# Autodesk Inventor assembly: КВ33.044.000
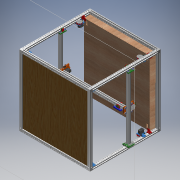
[picture p0: Inventor's stored thumbnail of the model, 180x180]
Saved by Autodesk Inventor 2019 (Build 230136000, 136)
## iProperties
Created: 2019-07-15
Part Number: КВ33.044.000
Material: Типовые
Document SubType Name: Assembly
Designer: Петров Иван
Description: Сортирующая ячейка
Author: Петров Иван
## Documents named in this file (14)
- E:\IVAN\Kvantoriada2019\optimal_gripper\hardware\КВ33.044.000 - Сортирующая ячейка.iam
- E:\IVAN\Kvantoriada2019\optimal_gripper\hardware\Стандартные изделия\Профиль станочный 30x30x740.ipt
- E:\IVAN\Kvantoriada2019\optimal_gripper\hardware\Стандартные изделия\Угол соединительный 30х30х30.ipt
- E:\IVAN\Kvantoriada2019\optimal_gripper\hardware\КВ33.044.001 - Дно.ipt
- E:\IVAN\Kvantoriada2019\optimal_gripper\hardware\КВ33.044.700 - Сборка деражтеля катка 6 мм.iam
- E:\IVAN\Kvantoriada2019\optimal_gripper\hardware\КВ33.044.400 -  Сборка сервомотора Dynamixel с крепление.iam
- E:\IVAN\Kvantoriada2019\optimal_gripper\hardware\КВ33.044.500 -  Сборка сервомотора Dynamixel с крепление обратный.iam
- E:\IVAN\Kvantoriada2019\optimal_gripper\hardware\КВ33.044.200 - Каретка оси Z.iam
- E:\IVAN\Kvantoriada2019\optimal_gripper\hardware\Стандартные изделия\Профиль станочный 30x30x717.ipt
- E:\IVAN\Kvantoriada2019\optimal_gripper\hardware\КВ33.044.300 - Каретка оси X.iam
- E:\IVAN\Kvantoriada2019\optimal_gripper\hardware\КВ33.044.003 - крепеж дна блока управления.ipt
- E:\IVAN\Kvantoriada2019\optimal_gripper\hardware\КВ33.044.100 - Блок управления.iam
- E:\IVAN\Kvantoriada2019\optimal_gripper\hardware\КВ33.044.005 - Крышка блока управления.ipt
- E:\IVAN\Kvantoriada2019\optimal_gripper\hardware\КВ33.044.600 - Каретка оси Y.iam
## Components (45 placed, 13 different names)
1. КВ33.044.001 - Дно:1 — Совмещение:65, Совмещение:66, Совмещение:67
2. Профиль станочный 30x30x740:1 — Заподлицо:9, Заподлицо:10, Совмещение:4, Заподлицо:12, Совмещение:9, Заподлицо:17
3. Профиль станочный 30x30x740:2 — Совмещение:3, Заподлицо:2, Заподлицо:3, Совмещение:66, Совмещение:67, Совмещение:105
4. Профиль станочный 30x30x740:3 — Совмещение:1, Заподлицо:1, Заподлицо:5, Заподлицо:6, Заподлицо:8, Совмещение:5, Совмещение:65, Совмещение:109
5. Профиль станочный 30x30x740:4 — Заподлицо:14, Совмещение:7, Заподлицо:16, Заподлицо:18, Заподлицо:19, Совмещение:10, Совмещение:100, Совмещение:113
6. Угол соединительный 30х30х30:1 — Совмещение:1, Совмещение:2, Совмещение:3, Заподлицо:1, Заподлицо:2, Заподлицо:3, Заподлицо:4, Заподлицо:5, Заподлицо:38
7. Угол соединительный 30х30х30:2 — Заподлицо:18, Заподлицо:19, Совмещение:10, Совмещение:11, Заподлицо:20, Заподлицо:21
8. Угол соединительный 30х30х30:3 — Заподлицо:6, Заподлицо:7, Заподлицо:8, Заподлицо:9, Заподлицо:10, Совмещение:4, Заподлицо:11, Совмещение:5, Совмещение:6
9. Угол соединительный 30х30х30:4 — Заподлицо:12, Заподлицо:13, Заподлицо:14, Заподлицо:15, Совмещение:7, Совмещение:8, Заподлицо:16, Совмещение:9, Заподлицо:17
10. Профиль станочный 30x30x740:9 — Заподлицо:7, Заподлицо:11, Совмещение:6, Совмещение:19, Заподлицо:36, Заподлицо:37, Совмещение:108, Заподлицо:46, Совмещение:139, Заподлицо:57, Совмещение:146, Совмещение:147, Совмещение:164, Совмещение:165
11. Профиль станочный 30x30x740:10 — Заподлицо:13, Заподлицо:15, Совмещение:8, Совмещение:112, Заподлицо:48, Совмещение:140, Заподлицо:58, Совмещение:148, Совмещение:149, Совмещение:173, Совмещение:175
12. Профиль станочный 30x30x740:11 — Совмещение:11, Заподлицо:20, Заподлицо:21, Совмещение:101, Заподлицо:42, Совмещение:134, Заподлицо:55, Совмещение:142, Совмещение:143, Совмещение:167, Совмещение:169
13. Профиль станочный 30x30x740:12 — Совмещение:2, Заподлицо:4, Заподлицо:38, Совмещение:104, Заподлицо:44, Совмещение:136, Заподлицо:56, Совмещение:144, Совмещение:145, Совмещение:170, Совмещение:171
14. Профиль станочный 30x30x740:15 — Совмещение:138, Совмещение:141
15. Профиль станочный 30x30x740:16 — Совмещение:135, Совмещение:137, Совмещение:177, Совмещение:179
16. Профиль станочный 30x30x740:17
17. Профиль станочный 30x30x740:18 — Совмещение:178, Совмещение:180
18. Угол соединительный 30х30х30:5
19. Угол соединительный 30х30х30:6
20. Угол соединительный 30х30х30:7 — Совмещение:19, Заподлицо:36, Заподлицо:37
21. Угол соединительный 30х30х30:8
22. КВ33.044.700 - Сборка деражтеля катка 6 мм:6 [sub-assembly] — Совмещение:100, Совмещение:101, Заподлицо:42
23. КВ33.044.700 - Сборка деражтеля катка 6 мм:7 [sub-assembly] — Совмещение:104, Заподлицо:44, Совмещение:105
24. КВ33.044.700 - Сборка деражтеля катка 6 мм:9 [sub-assembly] — Совмещение:108, Совмещение:109, Заподлицо:46
25. КВ33.044.700 - Сборка деражтеля катка 6 мм:10 [sub-assembly] — Совмещение:112, Заподлицо:48, Совмещение:113
26. КВ33.044.400 -  Сборка сервомотора Dynamixel с крепление:1 [sub-assembly] — Совмещение:134, Совмещение:135, Заподлицо:55, Совмещение:168
27. КВ33.044.500 -  Сборка сервомотора Dynamixel с крепление обратный:1 [sub-assembly] — Совмещение:136, Совмещение:137, Заподлицо:56, Совмещение:172
28. КВ33.044.400 -  Сборка сервомотора Dynamixel с крепление:2 [sub-assembly] — Совмещение:138, Совмещение:139, Заподлицо:57, Совмещение:166
29. КВ33.044.500 -  Сборка сервомотора Dynamixel с крепление обратный:2 [sub-assembly] — Совмещение:140, Заподлицо:58, Совмещение:141, Совмещение:174
30. КВ33.044.200 - Каретка оси Z:1 [sub-assembly] — Совмещение:142, Совмещение:143, Совмещение:152, Совмещение:153
31. КВ33.044.200 - Каретка оси Z:2 [sub-assembly] — Совмещение:148, Совмещение:149, Совмещение:156, Совмещение:157
32. КВ33.044.200 - Каретка оси Z:3 [sub-assembly] — Совмещение:146, Совмещение:147, Совмещение:154, Совмещение:155
33. КВ33.044.200 - Каретка оси Z:4 [sub-assembly] — Совмещение:144, Совмещение:145, Совмещение:150, Совмещение:151
34. Профиль станочный 30x30x717:1 — Совмещение:150, Совмещение:151, Совмещение:152, Совмещение:153, Совмещение:159, Заподлицо:60
35. Профиль станочный 30x30x717:2 — Совмещение:154, Совмещение:155, Совмещение:156, Совмещение:157, Совмещение:158, Заподлицо:59
36. КВ33.044.300 - Каретка оси X:1 [sub-assembly] — Совмещение:158, Заподлицо:59, Совмещение:163
37. КВ33.044.300 - Каретка оси X:2 [sub-assembly] — Совмещение:159, Заподлицо:60, Совмещение:160, Совмещение:161, Совмещение:162
38. Профиль станочный 30x30x717:3 — Совмещение:160, Совмещение:161, Совмещение:162, Совмещение:163, Совмещение:181, Совмещение:182
39. КВ33.044.003 - крепеж дна блока управления:1 — Совмещение:164, Совмещение:165, Совмещение:166
40. КВ33.044.003 - крепеж дна блока управления:2 — Совмещение:173, Совмещение:174, Совмещение:175
41. КВ33.044.003 - крепеж дна блока управления:3 — Совмещение:167, Совмещение:168, Совмещение:169
42. КВ33.044.003 - крепеж дна блока управления:4 — Совмещение:170, Совмещение:171, Совмещение:172, Совмещение:176
43. КВ33.044.100 - Блок управления:1 [sub-assembly] — Совмещение:176, Совмещение:177, Совмещение:178
44. КВ33.044.005 - Крышка блока управления:1 — Совмещение:179, Совмещение:180
45. КВ33.044.600 - Каретка оси Y:1 [sub-assembly] — Совмещение:181, Совмещение:182
## Relationships (127: Mate 79, Flush 48)
- Совмещение:1 [Mate]: Профиль станочный 30x30x740:3 ↔ Угол соединительный 30х30х30:1
- Совмещение:2 [Mate]: Угол соединительный 30х30х30:1 ↔ Профиль станочный 30x30x740:12
- Совмещение:3 [Mate]: Профиль станочный 30x30x740:2 ↔ Угол соединительный 30х30х30:1
- Заподлицо:1 [Flush]: Профиль станочный 30x30x740:3 ↔ Угол соединительный 30х30х30:1
- Заподлицо:2 [Flush]: Профиль станочный 30x30x740:2 ↔ Угол соединительный 30х30х30:1
- Заподлицо:3 [Flush]: Профиль станочный 30x30x740:2 ↔ Угол соединительный 30х30х30:1
- Заподлицо:4 [Flush]: Угол соединительный 30х30х30:1 ↔ Профиль станочный 30x30x740:12
- Заподлицо:5 [Flush]: Профиль станочный 30x30x740:3 ↔ Угол соединительный 30х30х30:1
- Заподлицо:6 [Flush]: Профиль станочный 30x30x740:3 ↔ Угол соединительный 30х30х30:3
- Заподлицо:7 [Flush]: Угол соединительный 30х30х30:3 ↔ Профиль станочный 30x30x740:9
- Заподлицо:8 [Flush]: Профиль станочный 30x30x740:3 ↔ Угол соединительный 30х30х30:3
- Заподлицо:9 [Flush]: Профиль станочный 30x30x740:1 ↔ Угол соединительный 30х30х30:3
- Заподлицо:10 [Flush]: Профиль станочный 30x30x740:1 ↔ Угол соединительный 30х30х30:3
- Совмещение:4 [Mate]: Профиль станочный 30x30x740:1 ↔ Угол соединительный 30х30х30:3
- Заподлицо:11 [Flush]: Угол соединительный 30х30х30:3 ↔ Профиль станочный 30x30x740:9
- Совмещение:5 [Mate]: Профиль станочный 30x30x740:3 ↔ Угол соединительный 30х30х30:3
- Совмещение:6 [Mate]: Угол соединительный 30х30х30:3 ↔ Профиль станочный 30x30x740:9
- Заподлицо:12 [Flush]: Профиль станочный 30x30x740:1 ↔ Угол соединительный 30х30х30:4
- Заподлицо:13 [Flush]: Угол соединительный 30х30х30:4 ↔ Профиль станочный 30x30x740:10
- Заподлицо:14 [Flush]: Профиль станочный 30x30x740:4 ↔ Угол соединительный 30х30х30:4
- Заподлицо:15 [Flush]: Угол соединительный 30х30х30:4 ↔ Профиль станочный 30x30x740:10
- Совмещение:7 [Mate]: Профиль станочный 30x30x740:4 ↔ Угол соединительный 30х30х30:4
- Совмещение:8 [Mate]: Угол соединительный 30х30х30:4 ↔ Профиль станочный 30x30x740:10
- Заподлицо:16 [Flush]: Профиль станочный 30x30x740:4 ↔ Угол соединительный 30х30х30:4
- Совмещение:9 [Mate]: Профиль станочный 30x30x740:1 ↔ Угол соединительный 30х30х30:4
- Заподлицо:17 [Flush]: Профиль станочный 30x30x740:1 ↔ Угол соединительный 30х30х30:4
- Заподлицо:18 [Flush]: Профиль станочный 30x30x740:4 ↔ Угол соединительный 30х30х30:2
- Заподлицо:19 [Flush]: Профиль станочный 30x30x740:4 ↔ Угол соединительный 30х30х30:2
- Совмещение:10 [Mate]: Профиль станочный 30x30x740:4 ↔ Угол соединительный 30х30х30:2
- Совмещение:11 [Mate]: Угол соединительный 30х30х30:2 ↔ Профиль станочный 30x30x740:11
- Заподлицо:20 [Flush]: Угол соединительный 30х30х30:2 ↔ Профиль станочный 30x30x740:11
- Заподлицо:21 [Flush]: Угол соединительный 30х30х30:2 ↔ Профиль станочный 30x30x740:11
- [Mate]: Профиль станочный 30x30x740:17 ↔ Угол соединительный 30х30х30:5
- [Mate]: Профиль станочный 30x30x740:16 ↔ Угол соединительный 30х30х30:5
- [Flush]: Профиль станочный 30x30x740:17 ↔ Угол соединительный 30х30х30:5
- [Flush]: Профиль станочный 30x30x740:16 ↔ Угол соединительный 30х30х30:5
- [Flush]: Профиль станочный 30x30x740:16 ↔ Угол соединительный 30х30х30:5
- [Flush]: Профиль станочный 30x30x740:17 ↔ Угол соединительный 30х30х30:5
- [Flush]: Профиль станочный 30x30x740:17 ↔ Угол соединительный 30х30х30:7
- [Flush]: Профиль станочный 30x30x740:17 ↔ Угол соединительный 30х30х30:7
- [Flush]: Профиль станочный 30x30x740:15 ↔ Угол соединительный 30х30х30:7
- [Flush]: Профиль станочный 30x30x740:15 ↔ Угол соединительный 30х30х30:7
- [Mate]: Профиль станочный 30x30x740:15 ↔ Угол соединительный 30х30х30:7
- [Mate]: Профиль станочный 30x30x740:17 ↔ Угол соединительный 30х30х30:7
- [Flush]: Профиль станочный 30x30x740:15 ↔ Угол соединительный 30х30х30:8
- [Flush]: Профиль станочный 30x30x740:18 ↔ Угол соединительный 30х30х30:8
- [Mate]: Профиль станочный 30x30x740:18 ↔ Угол соединительный 30х30х30:8
- [Flush]: Профиль станочный 30x30x740:18 ↔ Угол соединительный 30х30х30:8
- [Mate]: Профиль станочный 30x30x740:15 ↔ Угол соединительный 30х30х30:8
- [Flush]: Профиль станочный 30x30x740:15 ↔ Угол соединительный 30х30х30:8
- [Flush]: Профиль станочный 30x30x740:18 ↔ Угол соединительный 30х30х30:6
- [Flush]: Профиль станочный 30x30x740:18 ↔ Угол соединительный 30х30х30:6
- [Mate]: Профиль станочный 30x30x740:18 ↔ Угол соединительный 30х30х30:6
- Совмещение:19 [Mate]: Профиль станочный 30x30x740:9 ↔ Угол соединительный 30х30х30:7
- Заподлицо:36 [Flush]: Профиль станочный 30x30x740:9 ↔ Угол соединительный 30х30х30:7
- Заподлицо:37 [Flush]: Профиль станочный 30x30x740:9 ↔ Угол соединительный 30х30х30:7
- Заподлицо:38 [Flush]: Угол соединительный 30х30х30:1 ↔ Профиль станочный 30x30x740:12
- Совмещение:65 [Mate]: КВ33.044.001 - Дно:1 ↔ Профиль станочный 30x30x740:3
- Совмещение:66 [Mate]: КВ33.044.001 - Дно:1 ↔ Профиль станочный 30x30x740:2
- Совмещение:67 [Mate]: КВ33.044.001 - Дно:1 ↔ Профиль станочный 30x30x740:2
- Совмещение:100 [Mate]: Профиль станочный 30x30x740:4 ↔ КВ33.044.700 - Сборка деражтеля катка 6 мм:6
- Совмещение:101 [Mate]: Профиль станочный 30x30x740:11 ↔ КВ33.044.700 - Сборка деражтеля катка 6 мм:6
- Заподлицо:42 [Flush]: Профиль станочный 30x30x740:11 ↔ КВ33.044.700 - Сборка деражтеля катка 6 мм:6
- Совмещение:104 [Mate]: Профиль станочный 30x30x740:12 ↔ КВ33.044.700 - Сборка деражтеля катка 6 мм:7
- Заподлицо:44 [Flush]: Профиль станочный 30x30x740:12 ↔ КВ33.044.700 - Сборка деражтеля катка 6 мм:7
- Совмещение:105 [Mate]: Профиль станочный 30x30x740:2 ↔ КВ33.044.700 - Сборка деражтеля катка 6 мм:7
- Совмещение:108 [Mate]: Профиль станочный 30x30x740:9 ↔ КВ33.044.700 - Сборка деражтеля катка 6 мм:9
- Совмещение:109 [Mate]: Профиль станочный 30x30x740:3 ↔ КВ33.044.700 - Сборка деражтеля катка 6 мм:9
- Заподлицо:46 [Flush]: Профиль станочный 30x30x740:9 ↔ КВ33.044.700 - Сборка деражтеля катка 6 мм:9
- Совмещение:112 [Mate]: Профиль станочный 30x30x740:10 ↔ КВ33.044.700 - Сборка деражтеля катка 6 мм:10
- Заподлицо:48 [Flush]: Профиль станочный 30x30x740:10 ↔ КВ33.044.700 - Сборка деражтеля катка 6 мм:10
- Совмещение:113 [Mate]: Профиль станочный 30x30x740:4 ↔ КВ33.044.700 - Сборка деражтеля катка 6 мм:10
- Совмещение:134 [Mate]: Профиль станочный 30x30x740:11 ↔ КВ33.044.400 -  Сборка сервомотора Dynamixel с крепление:1
- Совмещение:135 [Mate] (130 mm): Профиль станочный 30x30x740:16 ↔ КВ33.044.400 -  Сборка сервомотора Dynamixel с крепление:1
- Заподлицо:55 [Flush]: Профиль станочный 30x30x740:11 ↔ КВ33.044.400 -  Сборка сервомотора Dynamixel с крепление:1
- Совмещение:136 [Mate]: Профиль станочный 30x30x740:12 ↔ КВ33.044.500 -  Сборка сервомотора Dynamixel с крепление обратный:1
- Совмещение:137 [Mate] (130 mm): Профиль станочный 30x30x740:16 ↔ КВ33.044.500 -  Сборка сервомотора Dynamixel с крепление обратный:1
- Заподлицо:56 [Flush]: Профиль станочный 30x30x740:12 ↔ КВ33.044.500 -  Сборка сервомотора Dynamixel с крепление обратный:1
- Совмещение:138 [Mate] (130 mm): Профиль станочный 30x30x740:15 ↔ КВ33.044.400 -  Сборка сервомотора Dynamixel с крепление:2
- Совмещение:139 [Mate]: Профиль станочный 30x30x740:9 ↔ КВ33.044.400 -  Сборка сервомотора Dynamixel с крепление:2
- Заподлицо:57 [Flush]: Профиль станочный 30x30x740:9 ↔ КВ33.044.400 -  Сборка сервомотора Dynamixel с крепление:2
- Совмещение:140 [Mate]: Профиль станочный 30x30x740:10 ↔ КВ33.044.500 -  Сборка сервомотора Dynamixel с крепление обратный:2
- Заподлицо:58 [Flush]: Профиль станочный 30x30x740:10 ↔ КВ33.044.500 -  Сборка сервомотора Dynamixel с крепление обратный:2
- Совмещение:141 [Mate] (130 mm): Профиль станочный 30x30x740:15 ↔ КВ33.044.500 -  Сборка сервомотора Dynamixel с крепление обратный:2
- Совмещение:142 [Mate] (1.5 mm): Профиль станочный 30x30x740:11 ↔ КВ33.044.200 - Каретка оси Z:1
- Совмещение:143 [Mate] (1.02 mm): Профиль станочный 30x30x740:11 ↔ КВ33.044.200 - Каретка оси Z:1
- Совмещение:144 [Mate] (1.5 mm): Профиль станочный 30x30x740:12 ↔ КВ33.044.200 - Каретка оси Z:4
- Совмещение:145 [Mate] (1.02 mm): Профиль станочный 30x30x740:12 ↔ КВ33.044.200 - Каретка оси Z:4
- Совмещение:146 [Mate] (1.5 mm): Профиль станочный 30x30x740:9 ↔ КВ33.044.200 - Каретка оси Z:3
- Совмещение:147 [Mate] (1.02 mm): Профиль станочный 30x30x740:9 ↔ КВ33.044.200 - Каретка оси Z:3
- Совмещение:148 [Mate] (1.5 mm): Профиль станочный 30x30x740:10 ↔ КВ33.044.200 - Каретка оси Z:2
- Совмещение:149 [Mate] (1.02 mm): Профиль станочный 30x30x740:10 ↔ КВ33.044.200 - Каретка оси Z:2
- Совмещение:150 [Mate]: КВ33.044.200 - Каретка оси Z:4 ↔ Профиль станочный 30x30x717:1
- Совмещение:151 [Mate]: КВ33.044.200 - Каретка оси Z:4 ↔ Профиль станочный 30x30x717:1
- Совмещение:152 [Mate]: КВ33.044.200 - Каретка оси Z:1 ↔ Профиль станочный 30x30x717:1
- Совмещение:153 [Mate]: КВ33.044.200 - Каретка оси Z:1 ↔ Профиль станочный 30x30x717:1
- Совмещение:154 [Mate]: КВ33.044.200 - Каретка оси Z:3 ↔ Профиль станочный 30x30x717:2
- Совмещение:155 [Mate]: КВ33.044.200 - Каретка оси Z:3 ↔ Профиль станочный 30x30x717:2
- Совмещение:156 [Mate]: КВ33.044.200 - Каретка оси Z:2 ↔ Профиль станочный 30x30x717:2
- Совмещение:157 [Mate]: КВ33.044.200 - Каретка оси Z:2 ↔ Профиль станочный 30x30x717:2
- Совмещение:158 [Mate] (1.5 mm): Профиль станочный 30x30x717:2 ↔ КВ33.044.300 - Каретка оси X:1
- Заподлицо:59 [Flush] (-19.235 mm): Профиль станочный 30x30x717:2 ↔ КВ33.044.300 - Каретка оси X:1
- Совмещение:159 [Mate] (1.5 mm): Профиль станочный 30x30x717:1 ↔ КВ33.044.300 - Каретка оси X:2
- Заподлицо:60 [Flush] (-19.235 mm): Профиль станочный 30x30x717:1 ↔ КВ33.044.300 - Каретка оси X:2
- Совмещение:160 [Mate]: КВ33.044.300 - Каретка оси X:2 ↔ Профиль станочный 30x30x717:3
- Совмещение:161 [Mate]: КВ33.044.300 - Каретка оси X:2 ↔ Профиль станочный 30x30x717:3
- Совмещение:162 [Mate]: КВ33.044.300 - Каретка оси X:2 ↔ Профиль станочный 30x30x717:3
- Совмещение:163 [Mate]: КВ33.044.300 - Каретка оси X:1 ↔ Профиль станочный 30x30x717:3
- Совмещение:164 [Mate]: Профиль станочный 30x30x740:9 ↔ КВ33.044.003 - крепеж дна блока управления:1
- Совмещение:165 [Mate]: Профиль станочный 30x30x740:9 ↔ КВ33.044.003 - крепеж дна блока управления:1
- Совмещение:166 [Mate] (10 mm): КВ33.044.400 -  Сборка сервомотора Dynamixel с крепление:2 ↔ КВ33.044.003 - крепеж дна блока управления:1
- Совмещение:167 [Mate]: Профиль станочный 30x30x740:11 ↔ КВ33.044.003 - крепеж дна блока управления:3
- Совмещение:168 [Mate] (10 mm): КВ33.044.400 -  Сборка сервомотора Dynamixel с крепление:1 ↔ КВ33.044.003 - крепеж дна блока управления:3
- Совмещение:169 [Mate]: Профиль станочный 30x30x740:11 ↔ КВ33.044.003 - крепеж дна блока управления:3
- Совмещение:170 [Mate]: Профиль станочный 30x30x740:12 ↔ КВ33.044.003 - крепеж дна блока управления:4
- Совмещение:171 [Mate]: Профиль станочный 30x30x740:12 ↔ КВ33.044.003 - крепеж дна блока управления:4
- Совмещение:172 [Mate] (10 mm): КВ33.044.500 -  Сборка сервомотора Dynamixel с крепление обратный:1 ↔ КВ33.044.003 - крепеж дна блока управления:4
- Совмещение:173 [Mate]: Профиль станочный 30x30x740:10 ↔ КВ33.044.003 - крепеж дна блока управления:2
- Совмещение:174 [Mate] (10 mm): КВ33.044.500 -  Сборка сервомотора Dynamixel с крепление обратный:2 ↔ КВ33.044.003 - крепеж дна блока управления:2
- Совмещение:175 [Mate]: Профиль станочный 30x30x740:10 ↔ КВ33.044.003 - крепеж дна блока управления:2
- Совмещение:176 [Mate]: КВ33.044.003 - крепеж дна блока управления:4 ↔ КВ33.044.100 - Блок управления:1
- Совмещение:177 [Mate]: Профиль станочный 30x30x740:16 ↔ КВ33.044.100 - Блок управления:1
- Совмещение:178 [Mate]: Профиль станочный 30x30x740:18 ↔ КВ33.044.100 - Блок управления:1
- Совмещение:179 [Mate]: Профиль станочный 30x30x740:16 ↔ КВ33.044.005 - Крышка блока управления:1
- Совмещение:180 [Mate]: Профиль станочный 30x30x740:18 ↔ КВ33.044.005 - Крышка блока управления:1
- Совмещение:181 [Mate] (1.5 mm): Профиль станочный 30x30x717:3 ↔ КВ33.044.600 - Каретка оси Y:1
- Совмещение:182 [Mate] (1.02 mm): Профиль станочный 30x30x717:3 ↔ КВ33.044.600 - Каретка оси Y:1
## Named parameters: d91_d80 = 0 mm, d92_d82 = 0 mm, d93_d83 = 0 mm, d94_d84 = 0 mm, d95_d85 = 0 mm, d96_d86 = 0 mm, d97_d87 = 0 mm, d98_d66 = 0 mm, d99_d67 = 0 mm, d100_d69 = 0 mm, d101_d70 = 0 mm, d102_d71 = 0 mm, d103_d72 = 0 mm, d104_d74 = 0 mm, d105_d76 = 0 mm, d106_d78 = 0 mm, d107_d59 = 0 mm, d108_d61 = 0 mm, d109_d62 = 0 mm, d110_d63 = 0 mm, d111_d64 = 0 mm
